# Autodesk Inventor assembly: MBD_Rdownframe
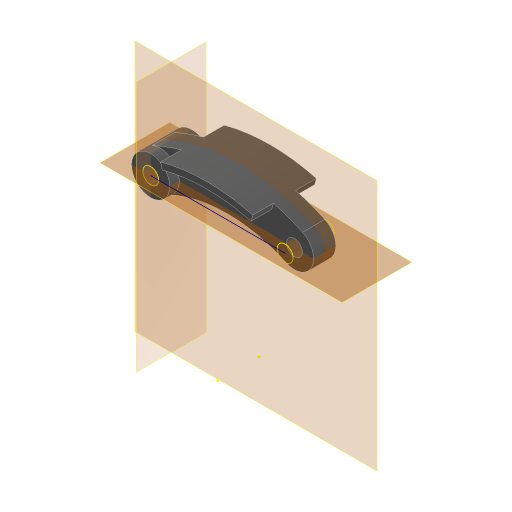
[picture p0: Inventor's stored thumbnail of the model, 512x512]
Saved by Autodesk Inventor 2023 (Build 270158000, 158)
## iProperties
Created: 2022-06-22
Part Number: MBD_Rdownframe
Document SubType Name: Assembly
Designer: BioRoLaT470S
Mass: 65.354 g
Surface Area: 170.529 cm^2
Volume: 36.1072 cm^3
Density: 1.81 g/cm^3
Author: BioRoLaT470S
## Documents named in this file (2)
- C:\Users\guanlunlu\Desktop\MBD_CORGI\CAD\MBD_Rdownframe.iam
- C:\Users\guanlunlu\Desktop\MBD_CORGI\R100_properties\組合檔_v4\下框1.ipt
## Components (1 placed, 1 different names)
1. 下框1:1 — Mate:1, Mate:2, Flush:1
## Relationships (3: Mate 2, Flush 1)
- Mate:1: 下框1:1
- Mate:2: 下框1:1
- Flush:1: 下框1:1
